# Autodesk Inventor assembly: Tail
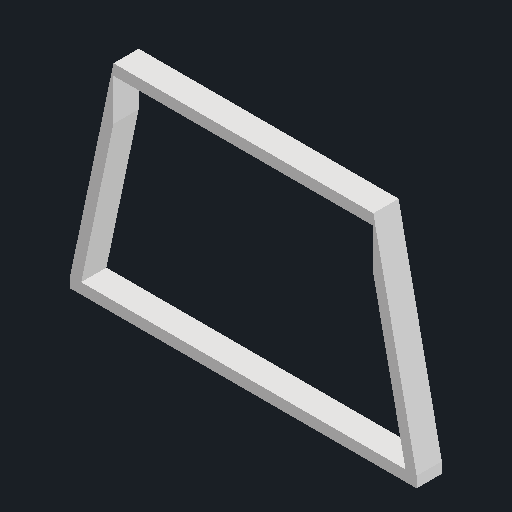
[picture p0: Inventor's stored thumbnail of the model, 512x512]
Saved by Autodesk Inventor 2026 (Build 300175000, 175)
## iProperties
Created: 2025-09-08
Part Number: Tail
Document SubType Name: Assembly
Designer: trott
Author: trott
## Documents named in this file (4)
- C:\Users\trott\Documents\UofSC-ASME-Tiger-Burn-Design-2025\CAD\Tail\Struct_tail.iam
- C:\Users\trott\Documents\UofSC-ASME-Tiger-Burn-Design-2025\CAD\Tail\2x4x48.ipt
- C:\Users\trott\Documents\UofSC-ASME-Tiger-Burn-Design-2025\CAD\Tail\S_2x4x29.334.ipt
- C:\Users\trott\Documents\UofSC-ASME-Tiger-Burn-Design-2025\CAD\Tail\2x4x36.ipt
## Components (4 placed, 3 different names)
1. 2x4x48:1 — Mate:1, Mate:2, Mate:3, Mate:4
2. S_2x4x29.334:1 — Mate:1, Mate:2
3. S_2x4x29.334:2 — Mate:3, Mate:4, Mate:5, Mate:6
4. 2x4x36:1 — Mate:5, Mate:6
## Relationships (6: Mate 6)
- Mate:1: 2x4x48:1 ↔ S_2x4x29.334:1
- Mate:2: 2x4x48:1 ↔ S_2x4x29.334:1
- Mate:3: 2x4x48:1 ↔ S_2x4x29.334:2
- Mate:4: 2x4x48:1 ↔ S_2x4x29.334:2
- Mate:5: S_2x4x29.334:2 ↔ 2x4x36:1
- Mate:6: S_2x4x29.334:2 ↔ 2x4x36:1
